# Autodesk Inventor assembly: VDPillar_A
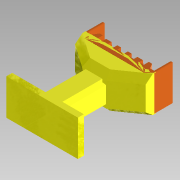
[picture p0: Inventor's stored thumbnail of the model, 180x180]
Saved by Autodesk Inventor 2021 (Build 250183000, 183)
## iProperties
Created: 2021-03-10
Part Number: VDPillar_A
Document SubType Name: Assembly
Designer: kumagai
Author: kumagai
## Documents named in this file (3)
- X:\Develop\CAD\PlaRails\ViaductPillar\VDPillar_A.iam
- X:\Develop\CAD\PlaRails\ViaductPillar\PillarTopVD.ipt
- X:\Develop\CAD\PlaRails\ViaductPillar\VDPillar_A.ipt
## Components (2 placed, 2 different names)
1. PillarTopVD:1
2. VDPillar_A:1 — フラッシュ:1, フラッシュ:4, フラッシュ:5
## Relationships (3: Flush 3)
- フラッシュ:1 [Flush]: VDPillar_A:1
- フラッシュ:4 [Flush]: VDPillar_A:1
- フラッシュ:5 [Flush]: VDPillar_A:1
